# Autodesk Inventor assembly: 4138T551_Gas Spring
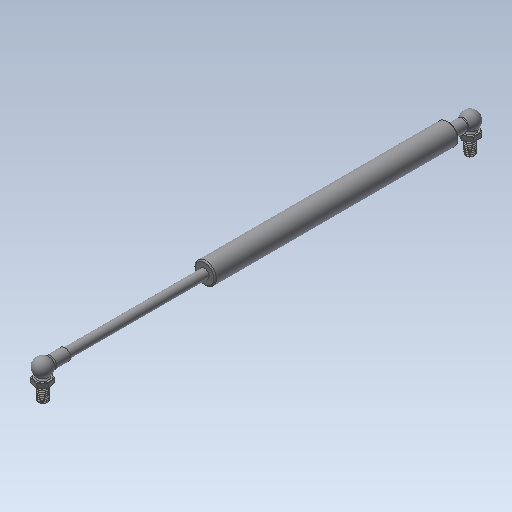
[picture p0: Inventor's stored thumbnail of the model, 512x512]
Saved by Autodesk Inventor 2020 (Build 240168000, 168)
## iProperties
Created: 2022-01-30
Part Number: 4138T551_Gas Spring
Document SubType Name: Assembly
Designer: mavericks
Mass: 63.4267 g
Surface Area: 259.564 cm^2
Volume: 63.4267 cm^3
Density: 1 g/cm^3
Author: mavericks
## Documents named in this file (6)
- T:\EIT\2022 Rapid React\COMMON PARTS\MCMASTER\Gas spring\4138T551_Gas Spring.iam
- T:\EIT\2022 Rapid React\COMMON PARTS\MCMASTER\Gas spring\Solid1_2.ipt
- T:\EIT\2022 Rapid React\COMMON PARTS\MCMASTER\Gas spring\Solid2_2.ipt
- T:\EIT\2022 Rapid React\COMMON PARTS\MCMASTER\Gas spring\Solid3_2.ipt
- T:\EIT\2022 Rapid React\COMMON PARTS\MCMASTER\Gas spring\Solid4_2.ipt
- T:\EIT\2022 Rapid React\COMMON PARTS\MCMASTER\Gas spring\Solid7_2.ipt
## Components (5 placed, 5 different names)
1. Solid1_2:1
2. Solid2_2:1 — Angle:1, Mate:6
3. Solid3_2:1 — Mate:1, Tangent:1, Mate:2, Mate:4
4. Solid4_2:1 — Mate:1
5. Solid7_2:1 — Tangent:1, Mate:2, Angle:1, Mate:4, Mate:5
## Relationships (7: Mate 5, Tangent 1, Angle 1)
- Mate:1: Solid3_2:1 ↔ Solid4_2:1
- Tangent:1: Solid3_2:1 ↔ Solid7_2:1
- Mate:2: Solid3_2:1 ↔ Solid7_2:1
- Angle:1 (180 deg): Solid2_2:1 ↔ Solid7_2:1
- Mate:4: Solid3_2:1 ↔ Solid7_2:1
- Mate:5: Solid7_2:1
- Mate:6: Solid2_2:1
